# Autodesk Inventor assembly: Инженерная графика
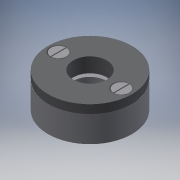
[picture p0: Inventor's stored thumbnail of the model, 180x180]
Saved by Autodesk Inventor 2019.3 (Build 233278000, 278)
## iProperties
Created: 2020-04-02
Part Number: Инженерная графика
Material: Типовые
Document SubType Name: Assembly
Designer: Admin
Mass: 143.908 g
Surface Area: 327.552 cm^2
Volume: 130.12 cm^3
Density: 1.10597 g/cm^3
Author: Admin
## Documents named in this file (4)
- D:\МГТУ Учеба\2 Семестр\Инжграф\Модуль 3\Инженерная графика.iam
- D:\МГТУ Учеба\2 Семестр\Инжграф\Модуль 3\Корпус.ipt
- D:\МГТУ Учеба\2 Семестр\Инжграф\Модуль 3\Крышка.ipt
- C:\Users\Admin\Documents\Inventor\Content Center Files\R2019\ru-RU\GOST 17475-80 (1)\Винт M8-6gx16 ГОСТ 17475-80.ipt
## Components (4 placed, 3 different names)
1. Корпус:1 — Жесткий:1
2. Крышка:1 — Жесткий:1
3. Винт ГОСТ 17475-80 M8 x 16:2
4. Винт ГОСТ 17475-80 M8 x 16:3
## Relationships (3: Mate 2, WeldJoint 1)
- Жесткий:1 [WeldJoint]: Корпус:1 ↔ Крышка:1
- [Mate]: Крышка:1 ↔ Винт ГОСТ 17475-80 M8 x 16:2
- [Mate]: Крышка:1 ↔ Винт ГОСТ 17475-80 M8 x 16:3
